# Autodesk Inventor assembly: FullAssembly
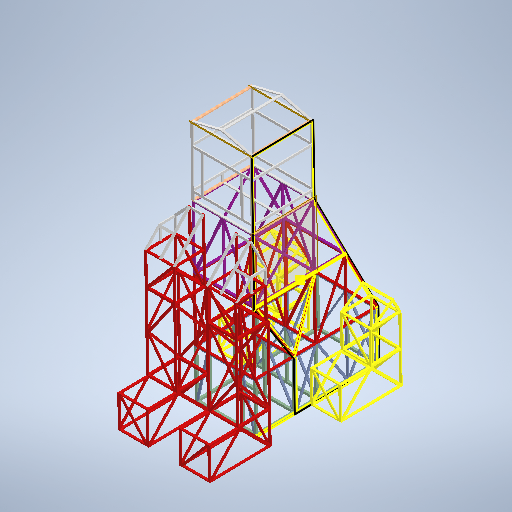
[picture p0: Inventor's stored thumbnail of the model, 512x512]
Saved by Autodesk Inventor 2025 (Build 290162000, 162)
## iProperties
Created: 2024-09-20
Part Number: FullAssembly
Document SubType Name: Assembly
Designer: localadmin
Author: localadmin
## Documents named in this file (13)
- C:\Users\localadmin\Documents\USCTigerBurn24\Tburn24\FullAssembly\FullAssembly.iam
- C:\Users\localadmin\Documents\USCTigerBurn24\Tburn24\layer0\Assembly1.iam
- C:\Users\localadmin\Documents\USCTigerBurn24\Tburn24\layer1\layer1.iam
- C:\Users\localadmin\Documents\USCTigerBurn24\Tburn24\layer2\layer2.iam
- C:\Users\localadmin\Documents\USCTigerBurn24\Tburn24\F_Legs1\B_Legs0.iam
- C:\Users\localadmin\Documents\USCTigerBurn24\Head.iam
- C:\Users\localadmin\Documents\USCTigerBurn24\Tburn24\Legs0\B_Legs0.iam
- C:\Users\localadmin\Documents\USCTigerBurn24\Tburn24\B_Legs1\B_Legs0.iam
- C:\Users\localadmin\Documents\USCTigerBurn24\Tburn24\F_Legs2\F_Legs2_MIR.iam
- C:\Users\localadmin\Documents\USCTigerBurn24\Tburn24\Legs0\B_Legs0_MIR.iam
- C:\Users\localadmin\Documents\USCTigerBurn24\Tburn24\F_Legs1\B_Legs0_MIR.iam
- C:\Users\localadmin\Documents\USCTigerBurn24\Tburn24\F_Legs2\F_Legs2_MIR_MIR.iam
- C:\Users\localadmin\Documents\USCTigerBurn24\Tburn24\FullAssembly\side wrap.ipt
## Components (15 placed, 9 different names)
1. Assembly1:1 [sub-assembly] — Mate:1, Flush:1, Flush:2, Mate:4, Flush:7, Flush:8, Flush:19, Flush:20, Mate:10, Flush:22, Flush:25
2. layer1:1 [sub-assembly] — Mate:1, Flush:1, Flush:2, Mate:2, Flush:3, Flush:4, Mate:13, Flush:23, Mate:14, Mate:17
3. layer2:1 [sub-assembly] — Mate:2, Flush:3, Flush:4, Mate:3, Flush:5, Flush:6, Flush:27, Flush:28
4. Head:1 [sub-assembly] — Mate:3, Flush:5, Flush:6
5. B_Legs0:1 [sub-assembly] — Mate:4, Flush:7, Flush:8, Mate:6, Flush:11, Flush:12
6. B_Legs0:2 [sub-assembly] — Mate:6, Flush:11, Flush:12, Mate:7, Flush:13, Flush:14
7. B_Legs0:3 [sub-assembly] — Mate:11, Mate:12, Flush:21, Mate:13, Flush:23, Mate:14, Flush:26
8. B_Legs0:6 [sub-assembly] — Mate:11, Mate:12, Flush:21, Flush:22
9. F_Legs2_MIR:1 [sub-assembly] — Mate:7, Flush:13, Flush:14
10. B_Legs0_MIR:1 [sub-assembly] — Flush:15, Flush:16, Mate:8, Flush:19, Flush:20, Mate:10
11. B_Legs0_MIR:2 [sub-assembly] — Flush:15, Flush:16, Mate:8, Flush:17, Flush:18, Mate:9
12. F_Legs2_MIR_MIR:1 [sub-assembly] — Flush:17, Flush:18, Mate:9
13. B_Legs0:7 [sub-assembly] — Mate:17, Flush:26
14. B_Legs0:8 [sub-assembly] — Flush:25
15. side wrap:1 — Flush:27, Flush:28
## Relationships (42: Flush 26, Mate 16)
- Mate:1: Assembly1:1 ↔ layer1:1
- Flush:1: Assembly1:1 ↔ layer1:1
- Flush:2: Assembly1:1 ↔ layer1:1
- Mate:2: layer1:1 ↔ layer2:1
- Flush:3: layer1:1 ↔ layer2:1
- Flush:4: layer1:1 ↔ layer2:1
- Mate:3: layer2:1 ↔ Head:1
- Flush:5: layer2:1 ↔ Head:1
- Flush:6: layer2:1 ↔ Head:1
- Mate:4: Assembly1:1 ↔ B_Legs0:1
- Flush:7: Assembly1:1 ↔ B_Legs0:1
- Flush:8: Assembly1:1 ↔ B_Legs0:1
- Mate:6: B_Legs0:1 ↔ B_Legs0:2
- Flush:11: B_Legs0:1 ↔ B_Legs0:2
- Flush:12: B_Legs0:1 ↔ B_Legs0:2
- Mate:7: B_Legs0:2 ↔ F_Legs2_MIR:1
- Flush:13: B_Legs0:2 ↔ F_Legs2_MIR:1
- Flush:14: B_Legs0:2 ↔ F_Legs2_MIR:1
- Flush:15: B_Legs0_MIR:1 ↔ B_Legs0_MIR:2
- Flush:16: B_Legs0_MIR:1 ↔ B_Legs0_MIR:2
- Mate:8: B_Legs0_MIR:1 ↔ B_Legs0_MIR:2
- Flush:17: B_Legs0_MIR:2 ↔ F_Legs2_MIR_MIR:1
- Flush:18: B_Legs0_MIR:2 ↔ F_Legs2_MIR_MIR:1
- Mate:9: B_Legs0_MIR:2 ↔ F_Legs2_MIR_MIR:1
- Flush:19: Assembly1:1 ↔ B_Legs0_MIR:1
- Flush:20: Assembly1:1 ↔ B_Legs0_MIR:1
- Mate:10: Assembly1:1 ↔ B_Legs0_MIR:1
- Mate:11: B_Legs0:3 ↔ B_Legs0:6
- Mate:12: B_Legs0:3 ↔ B_Legs0:6
- Flush:21: B_Legs0:3 ↔ B_Legs0:6
- Mate:13: layer1:1 ↔ B_Legs0:3
- Flush:22: Assembly1:1 ↔ B_Legs0:6
- Flush:23: layer1:1 ↔ B_Legs0:3
- Mate:14: layer1:1 ↔ B_Legs0:3
- [Mate]: B_Legs0:7 ↔ B_Legs0:8
- [Mate]: B_Legs0:7 ↔ B_Legs0:8
- [Flush]: B_Legs0:7 ↔ B_Legs0:8
- Flush:25: Assembly1:1 ↔ B_Legs0:8
- Mate:17: layer1:1 ↔ B_Legs0:7
- Flush:26: B_Legs0:3 ↔ B_Legs0:7
- Flush:27: layer2:1 ↔ side wrap:1
- Flush:28: layer2:1 ↔ side wrap:1
## Named parameters: d37_d30 = 0 mm, d38_d31 = 0 mm, d39_d32 = 0 mm
